# Autodesk Inventor assembly: Joystick
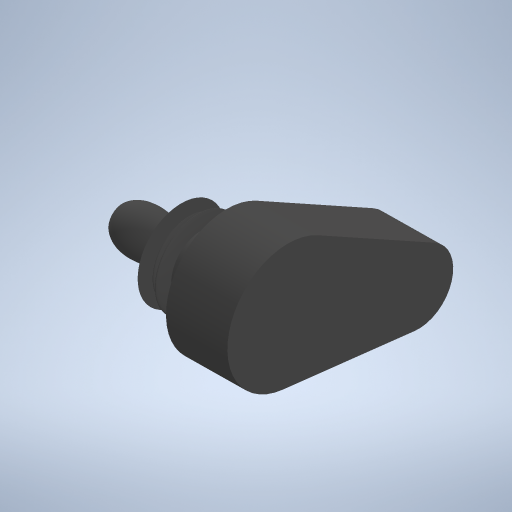
[picture p0: Inventor's stored thumbnail of the model, 512x512]
Saved by Autodesk Inventor 2023 (Build 270158000, 158)
## iProperties
Created: 2023-11-16
Part Number: Joystick
Document SubType Name: Assembly
Designer: DELL
Author: DELL
## Documents named in this file (3)
- D:\Rahul\IITGN\1st Year\EG Project\Joystick.iam
- D:\Rahul\IITGN\1st Year\EG Project\Joystick upper.ipt
- D:\Rahul\IITGN\1st Year\EG Project\Joystick base.ipt
## Components (2 placed, 2 different names)
1. Joystick upper:1 — Ball:1, Mate:1
2. Joystick base:1 — Ball:1
## Relationships (2: BallJoint 1, Mate 1)
- Ball:1: Joystick upper:1 ↔ Joystick base:1
- Mate:1: Joystick upper:1
